# Autodesk Inventor assembly: Assembly1
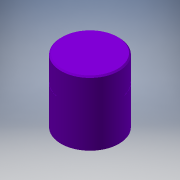
[picture p0: Inventor's stored thumbnail of the model, 180x180]
Saved by Autodesk Inventor 2019 (Build 230136000, 136)
## iProperties
Created: 2021-10-18
Part Number: Assembly1
Document SubType Name: Assembly
Designer: Mohamed Teleb
Author: Mohamed Teleb
## Documents named in this file (4)
- E:\Design of mechatronics 1\ThePart\Assembly1.iam
- E:\Design of mechatronics 1\ThePart\Part2.ipt
- E:\Design of mechatronics 1\ThePart\Part4.ipt
- E:\Design of mechatronics 1\ThePart\Magnet.ipt
## Components (4 placed, 3 different names)
1. Part2:1 — Mate:1, Rotational:1, Mate:2, Mate:3
2. Part4:1 — Mate:1, Rotational:1, Flush:1
3. Magnet:1 — Flush:1
4. Magnet:2 — Mate:2, Mate:3
## Relationships (5: Mate 3, RevoluteJoint 1, Flush 1)
- Mate:1: Part2:1 ↔ Part4:1
- Rotational:1 [RevoluteJoint]: Part2:1 ↔ Part4:1
- Flush:1: Part4:1 ↔ Magnet:1
- Mate:2: Part2:1 ↔ Magnet:2
- Mate:3: Part2:1 ↔ Magnet:2
